# Autodesk Inventor assembly: ESTRUCTURA_COMPLETA
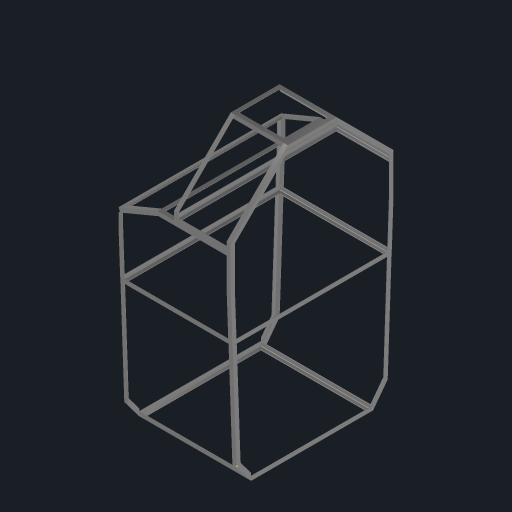
[picture p0: Inventor's stored thumbnail of the model, 512x512]
Saved by Autodesk Inventor 2024.3 (Build 283343000, 343)
## iProperties
Created: 2024-05-18
Part Number: ESTRUCTURA_COMPLETA
Material: Generic
Document SubType Name: Assembly
Designer: Niler
Author: Niler
## Documents named in this file (4)
- C:\Users\Niler\OneDrive\Escritorio\RECICLADOR\RECICLADOR_MODELO_3D\VERSION_3_COMPLETA\ESTRUCTURA\ESTRUCTURA_COMPLETA.iam
- C:\Users\Niler\OneDrive\Escritorio\RECICLADOR\RECICLADOR_MODELO_3D\VERSION_3_COMPLETA\ESTRUCTURA\ESTRUCTURA_V3_P1.iam
- C:\Users\Niler\OneDrive\Escritorio\RECICLADOR\RECICLADOR_MODELO_3D\VERSION_3_COMPLETA\ESTRUCTURA\ESTRUCTURA_V3_P2.iam
- C:\Users\Niler\OneDrive\Escritorio\RECICLADOR\RECICLADOR_MODELO_3D\VERSION_3_COMPLETA\ESTRUCTURA\ESTRUCTURA_V3_P3.iam
## Components (3 placed, 3 different names)
1. ESTRUCTURA_V3_P1:1 [sub-assembly] — Flush:5, Flush:6, Flush:7
2. ESTRUCTURA_V3_P2:1 [sub-assembly] — Mate:2, Flush:3, Flush:4, Flush:5, Flush:6, Flush:7
3. ESTRUCTURA_V3_P3:1 [sub-assembly] — Mate:2, Flush:3, Flush:4
## Relationships (6: Flush 5, Mate 1)
- Mate:2: ESTRUCTURA_V3_P2:1 ↔ ESTRUCTURA_V3_P3:1
- Flush:3: ESTRUCTURA_V3_P2:1 ↔ ESTRUCTURA_V3_P3:1
- Flush:4: ESTRUCTURA_V3_P2:1 ↔ ESTRUCTURA_V3_P3:1
- Flush:5: ESTRUCTURA_V3_P1:1 ↔ ESTRUCTURA_V3_P2:1
- Flush:6: ESTRUCTURA_V3_P1:1 ↔ ESTRUCTURA_V3_P2:1
- Flush:7: ESTRUCTURA_V3_P1:1 ↔ ESTRUCTURA_V3_P2:1
